# Autodesk Inventor assembly: S8x2
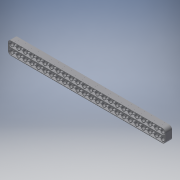
[picture p0: Inventor's stored thumbnail of the model, 180x180]
Saved by Autodesk Inventor 2019 (Build 230136000, 136)
## iProperties
Created: 2019-01-31
Part Number: S8x2
Document SubType Name: Assembly
Designer: Varga Daniel
Author: Varga Daniel
## Documents named in this file (3)
- C:\!_Dani\!_cloud\OneDrive\!_munka\Revolution\RevvyDemoKit\Structural parts\Straight Beams\S24x2.iam
- C:\!_Dani\!_cloud\OneDrive\!_munka\Revolution\RevvyDemoKit\Structural parts\Straight Beams\straight_beam_end_part_double.ipt
- C:\!_Dani\!_cloud\OneDrive\!_munka\Revolution\RevvyDemoKit\Structural parts\Straight Beams\straight_beam_inner_part_double.ipt
## Components (24 placed, 2 different names)
1. straight_beam_end_part_double:1 — Flush:8, Flush:9, Mate:2
2. straight_beam_end_part_double:2 — Flush:47, Flush:48, Mate:24
3. straight_beam_inner_part_double:1 — Flush:3, Flush:4, Flush:12, Flush:13, Mate:5, Mate:6
4. straight_beam_inner_part_double:2 — Flush:4, Flush:5, Flush:13, Flush:14, Mate:6, Mate:7
5. straight_beam_inner_part_double:3 — Flush:5, Flush:14, Mate:7, Flush:21, Flush:22, Mate:11
6. straight_beam_inner_part_double:4 — Flush:2, Flush:3, Flush:11, Flush:12, Mate:4, Mate:5
7. straight_beam_inner_part_double:5 — Flush:1, Flush:2, Flush:10, Flush:11, Mate:3, Mate:4
8. straight_beam_inner_part_double:6 — Flush:1, Flush:8, Flush:9, Mate:2, Flush:10, Mate:3
9. straight_beam_inner_part_double:7
10. straight_beam_inner_part_double:8
11. straight_beam_inner_part_double:9 — Flush:29, Flush:30, Mate:15
12. straight_beam_inner_part_double:10 — Flush:21, Flush:22, Mate:11
13. straight_beam_inner_part_double:11
14. straight_beam_inner_part_double:12
15. straight_beam_inner_part_double:13 — Flush:45, Flush:46, Mate:23
16. straight_beam_inner_part_double:14 — Flush:29, Flush:30, Mate:15
17. straight_beam_inner_part_double:15
18. straight_beam_inner_part_double:16
19. straight_beam_inner_part_double:17
20. straight_beam_inner_part_double:18 — Flush:45, Flush:46, Mate:23
21. straight_beam_inner_part_double:19
22. straight_beam_inner_part_double:20
23. straight_beam_inner_part_double:21 — Flush:47, Flush:48, Mate:24
24. straight_beam_inner_part_double:22
## Relationships (69: Flush 46, Mate 23)
- Flush:1: straight_beam_inner_part_double:5 ↔ straight_beam_inner_part_double:6
- Flush:2: straight_beam_inner_part_double:4 ↔ straight_beam_inner_part_double:5
- Flush:3: straight_beam_inner_part_double:1 ↔ straight_beam_inner_part_double:4
- Flush:4: straight_beam_inner_part_double:1 ↔ straight_beam_inner_part_double:2
- Flush:5: straight_beam_inner_part_double:2 ↔ straight_beam_inner_part_double:3
- Flush:8: straight_beam_end_part_double:1 ↔ straight_beam_inner_part_double:6
- Flush:9: straight_beam_end_part_double:1 ↔ straight_beam_inner_part_double:6
- Mate:2: straight_beam_end_part_double:1 ↔ straight_beam_inner_part_double:6
- Flush:10: straight_beam_inner_part_double:5 ↔ straight_beam_inner_part_double:6
- Flush:11: straight_beam_inner_part_double:4 ↔ straight_beam_inner_part_double:5
- Flush:12: straight_beam_inner_part_double:1 ↔ straight_beam_inner_part_double:4
- Flush:13: straight_beam_inner_part_double:1 ↔ straight_beam_inner_part_double:2
- Flush:14: straight_beam_inner_part_double:2 ↔ straight_beam_inner_part_double:3
- Mate:3: straight_beam_inner_part_double:5 ↔ straight_beam_inner_part_double:6
- Mate:4: straight_beam_inner_part_double:4 ↔ straight_beam_inner_part_double:5
- Mate:5: straight_beam_inner_part_double:1 ↔ straight_beam_inner_part_double:4
- Mate:6: straight_beam_inner_part_double:1 ↔ straight_beam_inner_part_double:2
- Mate:7: straight_beam_inner_part_double:2 ↔ straight_beam_inner_part_double:3
- [Flush]: straight_beam_inner_part_double:7 ↔ straight_beam_inner_part_double:10
- [Flush]: straight_beam_inner_part_double:7 ↔ straight_beam_inner_part_double:8
- [Flush]: straight_beam_inner_part_double:8 ↔ straight_beam_inner_part_double:9
- [Flush]: straight_beam_inner_part_double:7 ↔ straight_beam_inner_part_double:10
- [Flush]: straight_beam_inner_part_double:7 ↔ straight_beam_inner_part_double:8
- [Flush]: straight_beam_inner_part_double:8 ↔ straight_beam_inner_part_double:9
- [Mate]: straight_beam_inner_part_double:7 ↔ straight_beam_inner_part_double:10
- [Mate]: straight_beam_inner_part_double:7 ↔ straight_beam_inner_part_double:8
- [Mate]: straight_beam_inner_part_double:8 ↔ straight_beam_inner_part_double:9
- Flush:21: straight_beam_inner_part_double:3 ↔ straight_beam_inner_part_double:10
- Flush:22: straight_beam_inner_part_double:3 ↔ straight_beam_inner_part_double:10
- Mate:11: straight_beam_inner_part_double:3 ↔ straight_beam_inner_part_double:10
- [Flush]: straight_beam_inner_part_double:11 ↔ straight_beam_inner_part_double:14
- [Flush]: straight_beam_inner_part_double:11 ↔ straight_beam_inner_part_double:12
- [Flush]: straight_beam_inner_part_double:12 ↔ straight_beam_inner_part_double:13
- [Flush]: straight_beam_inner_part_double:11 ↔ straight_beam_inner_part_double:14
- [Flush]: straight_beam_inner_part_double:11 ↔ straight_beam_inner_part_double:12
- [Flush]: straight_beam_inner_part_double:12 ↔ straight_beam_inner_part_double:13
- [Mate]: straight_beam_inner_part_double:11 ↔ straight_beam_inner_part_double:14
- [Mate]: straight_beam_inner_part_double:11 ↔ straight_beam_inner_part_double:12
- [Mate]: straight_beam_inner_part_double:12 ↔ straight_beam_inner_part_double:13
- Flush:29: straight_beam_inner_part_double:9 ↔ straight_beam_inner_part_double:14
- Flush:30: straight_beam_inner_part_double:9 ↔ straight_beam_inner_part_double:14
- Mate:15: straight_beam_inner_part_double:9 ↔ straight_beam_inner_part_double:14
- [Flush]: straight_beam_inner_part_double:15 ↔ straight_beam_inner_part_double:18
- [Flush]: straight_beam_inner_part_double:15 ↔ straight_beam_inner_part_double:16
- [Flush]: straight_beam_inner_part_double:16 ↔ straight_beam_inner_part_double:17
- [Flush]: straight_beam_inner_part_double:15 ↔ straight_beam_inner_part_double:18
- [Flush]: straight_beam_inner_part_double:15 ↔ straight_beam_inner_part_double:16
- [Flush]: straight_beam_inner_part_double:16 ↔ straight_beam_inner_part_double:17
- [Mate]: straight_beam_inner_part_double:15 ↔ straight_beam_inner_part_double:18
- [Mate]: straight_beam_inner_part_double:15 ↔ straight_beam_inner_part_double:16
- [Mate]: straight_beam_inner_part_double:16 ↔ straight_beam_inner_part_double:17
- [Flush]: straight_beam_inner_part_double:19 ↔ straight_beam_inner_part_double:22
- [Flush]: straight_beam_inner_part_double:19 ↔ straight_beam_inner_part_double:20
- [Flush]: straight_beam_inner_part_double:20 ↔ straight_beam_inner_part_double:21
- [Flush]: straight_beam_inner_part_double:19 ↔ straight_beam_inner_part_double:22
- [Flush]: straight_beam_inner_part_double:19 ↔ straight_beam_inner_part_double:20
- [Flush]: straight_beam_inner_part_double:20 ↔ straight_beam_inner_part_double:21
- [Mate]: straight_beam_inner_part_double:19 ↔ straight_beam_inner_part_double:22
- [Mate]: straight_beam_inner_part_double:19 ↔ straight_beam_inner_part_double:20
- [Mate]: straight_beam_inner_part_double:20 ↔ straight_beam_inner_part_double:21
- [Flush]: straight_beam_inner_part_double:17 ↔ straight_beam_inner_part_double:22
- [Flush]: straight_beam_inner_part_double:17 ↔ straight_beam_inner_part_double:22
- [Mate]: straight_beam_inner_part_double:17 ↔ straight_beam_inner_part_double:22
- Flush:45: straight_beam_inner_part_double:13 ↔ straight_beam_inner_part_double:18
- Flush:46: straight_beam_inner_part_double:13 ↔ straight_beam_inner_part_double:18
- Mate:23: straight_beam_inner_part_double:13 ↔ straight_beam_inner_part_double:18
- Flush:47: straight_beam_end_part_double:2 ↔ straight_beam_inner_part_double:21
- Flush:48: straight_beam_end_part_double:2 ↔ straight_beam_inner_part_double:21
- Mate:24: straight_beam_end_part_double:2 ↔ straight_beam_inner_part_double:21
## Named parameters: d21_d13 = 0 mm, d22_d14 = 0 mm, d23_d15 = 0 mm, d24_d18 = 0 mm, d25_d19 = 0 mm, d26_d20 = 0 mm, d27_d2 = 0 mm, d28_d3 = 0 mm, d29_d4 = 0 mm, d36_d21_d13 = 0 mm, d37_d22_d14 = 0 mm, d38_d23_d15 = 0 mm, d39_d24_d18 = 0 mm, d40_d25_d19 = 0 mm, d41_d26_d20 = 0 mm, d42_d27_d2 = 0 mm, d43_d28_d3 = 0 mm, d44_d29_d4 = 0 mm, d51_d21_d13 = 0 mm, d52_d22_d14 = 0 mm, d53_d23_d15 = 0 mm, d54_d24_d18 = 0 mm, d55_d25_d19 = 0 mm, d56_d26_d20 = 0 mm, d57_d27_d2 = 0 mm, d58_d28_d3 = 0 mm, d59_d29_d4 = 0 mm, d60_d36_d21_d13 = 0 mm, d61_d37_d22_d14 = 0 mm, d62_d38_d23_d15 = 0 mm, d63_d39_d24_d18 = 0 mm, d64_d40_d25_d19 = 0 mm, d65_d41_d26_d20 = 0 mm, d66_d42_d27_d2 = 0 mm, d67_d43_d28_d3 = 0 mm, d68_d44_d29_d4 = 0 mm, d69_d45 = 0 mm, d70_d46 = 0 mm, d71_d47 = 0 mm
